# Autodesk Inventor assembly: rev6
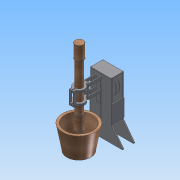
[picture p0: Inventor's stored thumbnail of the model, 180x180]
Saved by Autodesk Inventor 2015 (Build 190159000, 159)
## iProperties
Created: 2014-08-31
Part Number: rev6
Document SubType Name: Assembly
Designer: shohei
Author: shohei
## Documents named in this file (28)
- C:\Users\shohei\Documents\Inventor\FufuPounderGeared\rev6.iam
- C:\Users\shohei\Documents\Inventor\FufuPounderGeared\mortar2.ipt
- C:\Users\shohei\Documents\Inventor\FufuPounderGeared\sideplate.ipt
- C:\Users\shohei\Documents\Inventor\FufuPounderGeared\mainpulley.ipt
- C:\Users\shohei\Documents\Inventor\FufuPounderGeared\shaft5.ipt
- C:\Users\shohei\Documents\Inventor\FufuPounderGeared\drivelever.ipt
- C:\Users\shohei\Documents\Inventor\FufuPounderGeared\shaft7.ipt
- C:\Users\shohei\Documents\Inventor\FufuPounderGeared\globals.ipt
- C:\Users\shohei\Documents\Inventor\FufuPounderGeared\shaft8.ipt
- C:\Users\shohei\Documents\Inventor\FufuPounderGeared\shaft9.ipt
- C:\Users\shohei\Documents\Inventor\FufuPounderGeared\mallet_new.ipt
- C:\Users\shohei\Documents\Inventor\FufuPounderGeared\mallet_holder.ipt
- C:\Users\shohei\Documents\Inventor\FufuPounderGeared\mallet_sideplate.ipt
- C:\Users\shohei\Documents\Inventor\FufuPounderGeared\holderBlock.ipt
- C:\Users\shohei\Documents\Inventor\FufuPounderGeared\sideplate_top.ipt
- C:\Users\shohei\Documents\Inventor\FufuPounderGeared\shaft10.ipt
- C:\Users\shohei\Documents\Inventor\FufuPounderGeared\holderBlock2.ipt
- C:\Users\shohei\Documents\Inventor\FufuPounderGeared\gripsupport.ipt
- C:\Users\shohei\Documents\Inventor\FufuPounderGeared\M10washer.ipt
- C:\Users\shohei\Documents\Inventor\FufuPounderGeared\pulleyFlange.ipt
- C:\Users\shohei\Documents\Inventor\FufuPounderGeared\guardplate.ipt
- C:\Users\shohei\Documents\Inventor\FufuPounderGeared\drivepulleyAssembly.iam
- C:\Users\shohei\Documents\Inventor\FufuPounder\rev6\AIP\FEA\b5u4ebwdc.fins
- C:\Users\shohei\Documents\Inventor\FufuPounder\rev6\AIP\FEA\b5u4ebwdc.fsat
- C:\Users\shohei\Documents\Inventor\FufuPounder\rev6\AIP\FEA\b5u4ebwdc.ftes
- C:\Users\shohei\Documents\Inventor\FufuPounder\rev6\AIP\FEA\b5u4ebwdc.fwiz
- C:\Users\shohei\Documents\Inventor\FufuPounder\rev6\AIP\FEA\b5u4ebwgw.fmsh
- C:\Users\shohei\Documents\Inventor\FufuPounder\rev6\AIP\FEA\b5u4ebwgx.fres
## Components (46 placed, 21 different names)
1. mortar2:1 — Mate:1
2. sideplate:1 — Mate:2, Flush:1, Rotational:17, Flush:41, Flush:42, Mate:25, Mate:26, Flush:45
3. sideplate:2 — Mate:3, Flush:1, Rotational:10, Rotational:31, Slider:3, Mate:24, Flush:43, Flush:44, Flush:46, Slider:4
4. mainpulley:1 — Angle:1, Mate:23, Rotational:37, Rotational:39, Rigid:9
5. shaft5:2 — Cylindrical:8, Cylindrical:35, Rotational:38, Cylindrical:37
6. drivelever:1 — Cylindrical:37, Cylindrical:38, Cylindrical:39
7. shaft7:1 — Rotational:14, Rotational:19, Rotational:20, Slider:3, Rotational:40, Cylindrical:39
8. globals:1
9. mainpulley:2 — Rotational:33, Rotational:38, Rigid:10
10. shaft8:1 — Rotational:10, Rotational:33, Rigid:8
11. shaft9:2 — Cylindrical:4, Rigid:2, Rotational:22, Slider:4
12. mallet_new:1 — Rigid:1
13. mallet_holder:1 — Flush:3, Mate:5, Flush:4, Mate:6, Flush:5, Flush:6, Flush:9, Mate:7, Flush:10, Mate:8, Flush:11, Flush:12, Rigid:1, Flush:32
14. mallet_holder:2 — Flush:7, Mate:15, Flush:29, Flush:37
15. mallet_sideplate:1 — Flush:3, Mate:5, Flush:4, Flush:7, Mate:15, Flush:34, Flush:35, Mate:18, Mate:19, Flush:38, Flush:39
16. mallet_sideplate:2 — Flush:9, Mate:7, Flush:10
17. mallet_sideplate:3 — Mate:6, Flush:5, Flush:6, Mate:16, Mate:17, Flush:33, Flush:36
18. mallet_sideplate:4 — Mate:8, Flush:11, Flush:12, Flush:37
19. holderBlock:2 — Rotational:14, Cylindrical:4
20. sideplate_top:1 — Mate:24, Flush:41, Flush:42, Flush:43, Flush:46
21. shaft10:1 — Rotational:17, Rotational:30, Insert:1, Cylindrical:6, Rotational:39
22. holderBlock2:1 — Flush:28, Flush:40, Mate:20, Rotational:40
23. gripsupport:1 — Flush:32, Mate:17, Flush:33, Flush:40
24. gripsupport:2 — Flush:34, Flush:35, Mate:18, Mate:20
25. gripsupport:3 — Mate:19, Flush:38, Flush:39
26. gripsupport:4 — Mate:16, Flush:28, Flush:29, Flush:36
27. pulleyFlange:1 — Mate:23, Cylindrical:6
28. pulleyFlange:2 — Mate:21, Mate:22
29. pulleyFlange:3 — Rigid:8
30. guardplate:1 — Mate:25, Flush:44
31. guardplate:2 — Mate:26, Flush:45
32. drivepulleyAssembly:1 [sub-assembly] — Insert:1, Mate:21, Mate:22
33. M10washer:1
34. M10washer:2 — Rotational:19
35. M10washer:3 — Rigid:9
36. M10washer:4 — Cylindrical:8, Cylindrical:38
37. M10washer:5
38. M10washer:6 — Rotational:22
39. M10washer:7
40. M10washer:8 — Rigid:10
41. M10washer:9 — Rotational:20
42. M10washer:10 — Rigid:2
43. M10washer:11 — Cylindrical:35, Rotational:37
44. M10washer:14 — Rotational:31
45. M10washer:18 — Rotational:30
46. M10washer:22
## Relationships (75: Flush 27, Mate 19, RevoluteJoint 13, CylindricalJoint 7, WeldJoint 5, TranslationJoint 2, Angle 1, Insert 1)
- Mate:1: mortar2:1
- Mate:2: sideplate:1
- Mate:3: sideplate:2
- Flush:1: sideplate:1 ↔ sideplate:2
- Angle:1 (360 deg): mainpulley:1
- Rotational:10 [RevoluteJoint]: sideplate:2 ↔ shaft8:1
- Flush:3: mallet_holder:1 ↔ mallet_sideplate:1
- Mate:5: mallet_holder:1 ↔ mallet_sideplate:1
- Flush:4: mallet_holder:1 ↔ mallet_sideplate:1
- Mate:6: mallet_holder:1 ↔ mallet_sideplate:3
- Flush:5: mallet_holder:1 ↔ mallet_sideplate:3
- Flush:6: mallet_holder:1 ↔ mallet_sideplate:3
- Flush:7: mallet_holder:2 ↔ mallet_sideplate:1
- Flush:9: mallet_holder:1 ↔ mallet_sideplate:2
- Mate:7: mallet_holder:1 ↔ mallet_sideplate:2
- Flush:10: mallet_holder:1 ↔ mallet_sideplate:2
- Mate:8: mallet_holder:1 ↔ mallet_sideplate:4
- Flush:11: mallet_holder:1 ↔ mallet_sideplate:4
- Flush:12: mallet_holder:1 ↔ mallet_sideplate:4
- Rotational:14 [RevoluteJoint] (-30 mm): shaft7:1 ↔ holderBlock:2
- Cylindrical:4: shaft9:2 ↔ holderBlock:2
- Rotational:17 [RevoluteJoint] (-80 mm): sideplate:1 ↔ shaft10:1
- Mate:15: mallet_holder:2 ↔ mallet_sideplate:1
- Rigid:1 [WeldJoint]: mallet_new:1 ↔ mallet_holder:1
- Mate:16: mallet_sideplate:3 ↔ gripsupport:4
- Flush:28: holderBlock2:1 ↔ gripsupport:4
- Flush:29: mallet_holder:2 ↔ gripsupport:4
- Rotational:19 [RevoluteJoint] (-22 mm): shaft7:1 ↔ M10washer:2
- Rotational:20 [RevoluteJoint] (-50 mm): shaft7:1 ↔ M10washer:9
- Rigid:2 [WeldJoint] (-20 mm): shaft9:2 ↔ M10washer:10
- Rotational:22 [RevoluteJoint]: shaft9:2 ↔ M10washer:6
- Rotational:30 [RevoluteJoint] (-10 mm): shaft10:1 ↔ M10washer:18
- Rotational:31 [RevoluteJoint] (-2 mm): sideplate:2 ↔ M10washer:14
- Flush:32: mallet_holder:1 ↔ gripsupport:1
- Mate:17: mallet_sideplate:3 ↔ gripsupport:1
- Flush:33: mallet_sideplate:3 ↔ gripsupport:1
- Flush:34: mallet_sideplate:1 ↔ gripsupport:2
- Flush:35: mallet_sideplate:1 ↔ gripsupport:2
- Mate:18: mallet_sideplate:1 ↔ gripsupport:2
- Flush:36: mallet_sideplate:3 ↔ gripsupport:4
- Flush:37: mallet_holder:2 ↔ mallet_sideplate:4
- Mate:19: mallet_sideplate:1 ↔ gripsupport:3
- Flush:38: mallet_sideplate:1 ↔ gripsupport:3
- Flush:39: mallet_sideplate:1 ↔ gripsupport:3
- Flush:40: holderBlock2:1 ↔ gripsupport:1
- Mate:20: holderBlock2:1 ↔ gripsupport:2
- Insert:1: shaft10:1 ↔ drivepulleyAssembly:1
- Mate:21: pulleyFlange:2 ↔ drivepulleyAssembly:1
- Mate:22: pulleyFlange:2 ↔ drivepulleyAssembly:1
- Mate:23: mainpulley:1 ↔ pulleyFlange:1
- Cylindrical:6: shaft10:1 ↔ pulleyFlange:1
- Rotational:33 [RevoluteJoint]: mainpulley:2 ↔ shaft8:1
- Rigid:8 [WeldJoint] (20 mm): shaft8:1 ↔ pulleyFlange:3
- Cylindrical:8: shaft5:2 ↔ M10washer:4
- Cylindrical:35: shaft5:2 ↔ M10washer:11
- Rotational:37 [RevoluteJoint]: mainpulley:1 ↔ M10washer:11
- Rotational:38 [RevoluteJoint]: shaft5:2 ↔ mainpulley:2
- Slider:3 [TranslationJoint] (-40 mm): sideplate:2 ↔ shaft7:1
- Mate:24: sideplate:2 ↔ sideplate_top:1
- Flush:41: sideplate:1 ↔ sideplate_top:1
- Flush:42: sideplate:1 ↔ sideplate_top:1
- Flush:43: sideplate:2 ↔ sideplate_top:1
- Rotational:39 [RevoluteJoint]: mainpulley:1 ↔ shaft10:1
- Cylindrical:37: shaft5:2 ↔ drivelever:1
- Cylindrical:38: drivelever:1 ↔ M10washer:4
- Mate:25: sideplate:1 ↔ guardplate:1
- Flush:44: sideplate:2 ↔ guardplate:1
- Mate:26: sideplate:1 ↔ guardplate:2
- Flush:45: sideplate:1 ↔ guardplate:2
- Rotational:40 [RevoluteJoint]: shaft7:1 ↔ holderBlock2:1
- Flush:46: sideplate:2 ↔ sideplate_top:1
- Slider:4 [TranslationJoint] (40 mm): sideplate:2 ↔ shaft9:2
- Cylindrical:39: drivelever:1 ↔ shaft7:1
- Rigid:9 [WeldJoint]: mainpulley:1 ↔ M10washer:3
- Rigid:10 [WeldJoint]: mainpulley:2 ↔ M10washer:8
## Named parameters: sa_0 = 0, sa_1 = 3.2e-12, sa_2 = 10000
note: some values were not read from the file. Shown as the stored number, unit unknown: "sa_0", "sa_1", "sa_2".
